# Autodesk Inventor assembly: Wankel
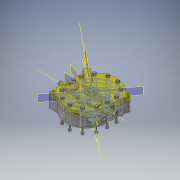
[picture p0: Inventor's stored thumbnail of the model, 180x180]
Saved by Autodesk Inventor 2019.4 (Build 234330000, 330)
## iProperties
Created: 2020-05-01
Part Number: Wankel
Document SubType Name: Assembly
Designer: Gabriel
Author: Gabriel
## Documents named in this file (9)
- C:\Users\Gabriel\Desktop\Teme Gac\MotorWankel\Wankel.iam
- C:\Users\Gabriel\Desktop\Teme Gac\MotorWankel\CapacSpate.ipt
- C:\Users\Gabriel\Desktop\Teme Gac\MotorWankel\StatorWankel.ipt
- C:\Users\Gabriel\Desktop\Teme Gac\MotorWankel\Arbore.ipt
- C:\Users\Gabriel\Desktop\Teme Gac\MotorWankel\SansRotor.iam
- C:\Users\Gabriel\Desktop\Teme Gac\MotorWankel\SansCapacFata.iam
- C:\Users\Gabriel\Desktop\Teme Gac\MotorWankel\Ans Suruburi Fixare.iam
- C:\Users\Gabriel\Desktop\Teme Gac\MotorWankel\Ans Piulite Fixare.iam
- C:\Users\Gabriel\Documents\Inventor\Content Center Files\R2019\en-US\ISO 6194 1  T 1\ISO 6194_1 - Type1 22 x 35 x 7.ipt
## Components (9 placed, 8 different names)
1. CapacSpate:1 — Mate:1, Mate:2, Angle:1, Mate:3, Mate:4, Mate:5, Mate:11
2. StatorWankel:1 — Mate:1, Mate:2, Angle:1, Unghi Animatie, Mate:8, Mate:10
3. Arbore:1 — Mate:3, Mate:4, Unghi Animatie, Mate:6, Mate:7, Rotation:1, Mate:9, Mate:12, Mate:14
4. SansRotor:1 [sub-assembly] — Mate:5, Mate:6, Mate:7, Rotation:1
5. SansCapacFata:1 [sub-assembly] — Mate:8, Mate:9, Mate:10, Mate:13
6. Ans Suruburi Fixare:1 [sub-assembly]
7. Ans Piulite Fixare:1 [sub-assembly]
8. ISO 6194/1 Type 1 Type1 22 x 35 x 7:1 — Mate:11, Mate:12
9. ISO 6194/1 Type 1 Type1 22 x 35 x 7:2 — Mate:13, Mate:14
## Relationships (19: Mate 14, Angle 2, Insert 2, RelateRotation 1)
- Mate:1: CapacSpate:1 ↔ StatorWankel:1
- Mate:2: CapacSpate:1 ↔ StatorWankel:1
- Angle:1 (0 deg): CapacSpate:1 ↔ StatorWankel:1
- Mate:3 (1 mm): CapacSpate:1 ↔ Arbore:1
- Mate:4: CapacSpate:1 ↔ Arbore:1
- Unghi Animatie [Angle] (1080 deg): StatorWankel:1 ↔ Arbore:1
- Mate:5: CapacSpate:1 ↔ SansRotor:1
- Mate:6: Arbore:1 ↔ SansRotor:1
- Mate:7: Arbore:1 ↔ SansRotor:1
- Rotation:1 [RelateRotation] (3 ul): Arbore:1 ↔ SansRotor:1
- Mate:8: StatorWankel:1 ↔ SansCapacFata:1
- Mate:9: Arbore:1 ↔ SansCapacFata:1
- Mate:10: StatorWankel:1 ↔ SansCapacFata:1
- [Insert]: SansCapacFata:1 ↔ Ans Suruburi Fixare:1
- [Insert]: CapacSpate:1 ↔ Ans Piulite Fixare:1
- Mate:11: CapacSpate:1 ↔ ISO 6194/1 Type 1 Type1 22 x 35 x 7:1
- Mate:12: Arbore:1 ↔ ISO 6194/1 Type 1 Type1 22 x 35 x 7:1
- Mate:13: SansCapacFata:1 ↔ ISO 6194/1 Type 1 Type1 22 x 35 x 7:2
- Mate:14: Arbore:1 ↔ ISO 6194/1 Type 1 Type1 22 x 35 x 7:2
